# Autodesk Inventor assembly: TB_Fullassemb
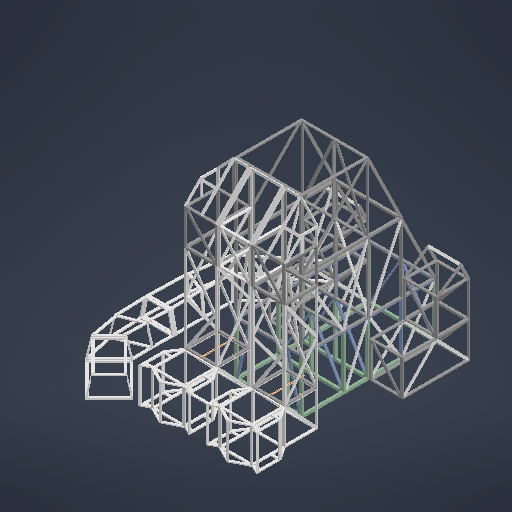
[picture p0: Inventor's stored thumbnail of the model, 512x512]
Saved by Autodesk Inventor 2026 (Build 300175000, 175)
## iProperties
Created: 2025-08-28
Part Number: TB_Fullassemb
Document SubType Name: Assembly
Designer: trott
Author: trott
## Documents named in this file (11)
- C:\Users\trott\Documents\UofSC-ASME-Tiger-Burn-Design-2025\CAD\Assembly\TB_Fullassemb.iam
- C:\Users\trott\Documents\UofSC-ASME-Tiger-Burn-Design-2025\CAD\Body\Base 01\Base 01.iam
- C:\Users\trott\Documents\UofSC-ASME-Tiger-Burn-Design-2025\CAD\Body\Base 02\Base 02.iam
- C:\Users\trott\Documents\UofSC-ASME-Tiger-Burn-Design-2025\CAD\Body\Base 03\Base 03.iam
- C:\Users\trott\Documents\UofSC-ASME-Tiger-Burn-Design-2025\CAD\Legs\Shoulder\Shoulder_L\Shoulder_L.iam
- C:\Users\trott\Documents\UofSC-ASME-Tiger-Burn-Design-2025\CAD\Legs\Shoulder\Shoulder_R\Shoulder_R.iam
- C:\Users\trott\Documents\UofSC-ASME-Tiger-Burn-Design-2025\CAD\Legs\Back Foot\B_Foot.iam
- C:\Users\trott\Documents\UofSC-ASME-Tiger-Burn-Design-2025\CAD\Legs\Back Leg\B_Leg.iam
- C:\Users\trott\Documents\UofSC-ASME-Tiger-Burn-Design-2025\CAD\Legs\Front Leg\F_Leg.iam
- C:\Users\trott\Documents\UofSC-ASME-Tiger-Burn-Design-2025\CAD\Legs\Front Foot\F_Foot.iam
- C:\Users\trott\Documents\UofSC-ASME-Tiger-Burn-Design-2025\CAD\Tail\Tail.iam
## Components (14 placed, 10 different names)
1. Base 01:1 [sub-assembly] — Mate:1, Flush:1, Flush:2, Flush:8, Mate:5, Flush:9, Mate:6, Flush:10, Flush:11, Flush:12, Mate:8, Flush:13
2. Base 02:1 [sub-assembly] — Mate:1, Flush:1, Flush:2, Mate:2, Flush:3, Flush:4, Mate:21, Mate:23
3. Base 03:1 [sub-assembly] — Mate:2, Flush:3, Flush:4, Flush:5, Flush:6, Mate:3, Mate:4, Flush:7, Mate:10, Flush:14, Mate:11, Mate:12, Mate:13, Mate:14, Flush:15
4. Shoulder_L:1 [sub-assembly] — Flush:5, Flush:6, Mate:3, Mate:10, Flush:14, Mate:11, Mate:20, Flush:26
5. Shoulder_R:1 [sub-assembly] — Mate:4, Flush:7, Mate:12, Mate:13, Mate:14, Flush:15, Mate:22, Flush:27
6. B_Foot:1 [sub-assembly] — Flush:8, Mate:5, Flush:9, Mate:7, Mate:19, Flush:24, Flush:25
7. B_Foot:2 [sub-assembly] — Mate:6, Flush:10, Flush:11, Mate:9
8. B_Leg:1 [sub-assembly] — Mate:7, Flush:12, Mate:8
9. B_Leg:2 [sub-assembly] — Mate:9, Flush:13
10. F_Foot:1 [sub-assembly] — Flush:29, Flush:31
11. F_Foot:2 [sub-assembly] — Flush:28, Flush:30
12. Tail:1 [sub-assembly] — Mate:19, Flush:24, Flush:25
13. F_Leg:3 [sub-assembly] — Mate:20, Mate:21, Flush:26, Flush:28, Flush:30
14. F_Leg:4 [sub-assembly] — Mate:22, Mate:23, Flush:27, Flush:29, Flush:31
## Relationships (42: Flush 23, Mate 19)
- Mate:1: Base 01:1 ↔ Base 02:1
- Flush:1: Base 01:1 ↔ Base 02:1
- Flush:2: Base 01:1 ↔ Base 02:1
- Mate:2: Base 02:1 ↔ Base 03:1
- Flush:3: Base 02:1 ↔ Base 03:1
- Flush:4: Base 02:1 ↔ Base 03:1
- Flush:5: Base 03:1 ↔ Shoulder_L:1
- Flush:6: Base 03:1 ↔ Shoulder_L:1
- Mate:3: Base 03:1 ↔ Shoulder_L:1
- Mate:4: Base 03:1 ↔ Shoulder_R:1
- Flush:7: Base 03:1 ↔ Shoulder_R:1
- Flush:8: Base 01:1 ↔ B_Foot:1
- Mate:5: Base 01:1 ↔ B_Foot:1
- Flush:9: Base 01:1 ↔ B_Foot:1
- Mate:6: Base 01:1 ↔ B_Foot:2
- Flush:10: Base 01:1 ↔ B_Foot:2
- Flush:11: Base 01:1 ↔ B_Foot:2
- Mate:7: B_Foot:1 ↔ B_Leg:1
- Flush:12: Base 01:1 ↔ B_Leg:1
- Mate:8: Base 01:1 ↔ B_Leg:1
- Mate:9: B_Foot:2 ↔ B_Leg:2
- Flush:13: Base 01:1 ↔ B_Leg:2
- Mate:10: Base 03:1 ↔ Shoulder_L:1
- Flush:14: Base 03:1 ↔ Shoulder_L:1
- Mate:11: Base 03:1 ↔ Shoulder_L:1
- Mate:12: Base 03:1 ↔ Shoulder_R:1
- Mate:13: Base 03:1 ↔ Shoulder_R:1
- Mate:14: Base 03:1 ↔ Shoulder_R:1
- Flush:15: Base 03:1 ↔ Shoulder_R:1
- Mate:19: B_Foot:1 ↔ Tail:1
- Flush:24: B_Foot:1 ↔ Tail:1
- Flush:25: B_Foot:1 ↔ Tail:1
- Mate:20: Shoulder_L:1 ↔ F_Leg:3
- Mate:21: Base 02:1 ↔ F_Leg:3
- Flush:26: Shoulder_L:1 ↔ F_Leg:3
- Mate:22: Shoulder_R:1 ↔ F_Leg:4
- Mate:23: Base 02:1 ↔ F_Leg:4
- Flush:27: Shoulder_R:1 ↔ F_Leg:4
- Flush:28: F_Foot:2 ↔ F_Leg:3
- Flush:29: F_Foot:1 ↔ F_Leg:4
- Flush:30: F_Foot:2 ↔ F_Leg:3
- Flush:31: F_Foot:1 ↔ F_Leg:4
